# Autodesk Inventor assembly: PowerTransmission
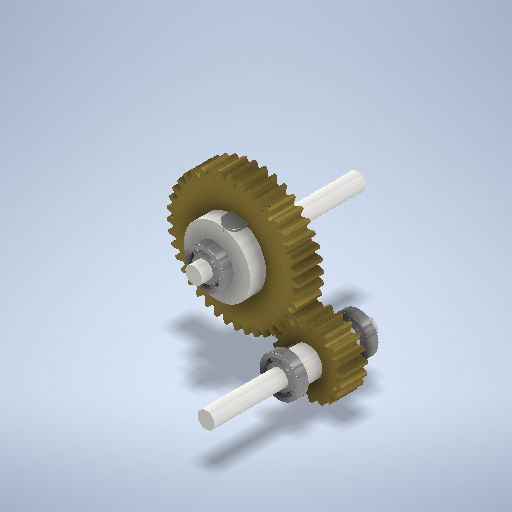
[picture p0: Inventor's stored thumbnail of the model, 512x512]
Saved by Autodesk Inventor 2025.2 (Build 292293000, 293)
## iProperties
Created: 2024-11-07
Part Number: PowerTransmission
Document SubType Name: Assembly
Designer: hongquan
Author: hongquan
## Documents named in this file (8)
- C:\Users\hongquan\Documents\GitHub\Optimal-Design-Robot\Inventor\PowerTransmission.iam
- C:\Users\hongquan\Documents\GitHub\Optimal-Design-Robot\Inventor\PowerTransmission\Design Accelerator\Spur Gears1.iam
- C:\Users\hongquan\Documents\GitHub\Optimal-Design-Robot\Inventor\PowerTransmission\Design Accelerator\Spur Gears2.iam
- C:\Users\hongquan\Documents\GitHub\Optimal-Design-Robot\Inventor\Shaft1.ipt
- C:\Users\hongquan\Documents\GitHub\Optimal-Design-Robot\Inventor\Shaft2.ipt
- C:\Users\hongquan\Documents\GitHub\Optimal-Design-Robot\Inventor\PowerTransmission\Design Accelerator\Key Connection1.iam
- C:\Users\hongquan\Documents\GitHub\Optimal-Design-Robot\Inventor\PowerTransmission\Design Accelerator\Key Connection3.iam
- C:\Users\hongquan\Documents\GitHub\Optimal-Design-Robot\Inventor\PowerTransmission\Design Accelerator\Bearing1.iam
## Components (10 placed, 4 different names)
1. Spur Gears:1 [sub-assembly]
2. Spur Gears:2 [sub-assembly] — Mate:1, Flush:1, Mate:4, Angle:2, Angle:4
3. Shaft:2 — Mate:2, Flush:1, Flush:2, Flush:3, Angle:1, Mate:5, Angle:2, Mate:11, Mate:12, Mate:13, Mate:14
4. Shaft:1 — Mate:4, Flush:2, Flush:4, Angle:3, Mate:6, Angle:4, Mate:7, Mate:8, Mate:9, Mate:10
5. Key Connection:1 [sub-assembly] — Flush:3, Angle:1, Mate:5
6. Key Connection:2 [sub-assembly] — Flush:4, Angle:3, Mate:6
7. Bearing:1 [sub-assembly] — Mate:7, Mate:8
8. Bearing:2 [sub-assembly] — Mate:11, Mate:12
9. Bearing:3 [sub-assembly] — Mate:13, Mate:14
10. Bearing:4 [sub-assembly] — Mate:9, Mate:10
## Relationships (21: Mate 13, Flush 4, Angle 4)
- Mate:1: Spur Gears:2
- Mate:2: Shaft:2
- Flush:1 (30 mm): Spur Gears:2 ↔ Shaft:2
- Mate:4: Spur Gears:2 ↔ Shaft:1
- Flush:2: Shaft:2 ↔ Shaft:1
- Flush:3: Shaft:2 ↔ Key Connection:1
- Angle:1 (355 deg): Shaft:2 ↔ Key Connection:1
- Mate:5: Shaft:2 ↔ Key Connection:1
- Angle:2 (124.6435 deg): Spur Gears:2 ↔ Shaft:2
- Flush:4 (10.1713 mm): Shaft:1 ↔ Key Connection:2
- Angle:3 (0 deg): Shaft:1 ↔ Key Connection:2
- Mate:6: Shaft:1 ↔ Key Connection:2
- Angle:4 (3.146 deg): Spur Gears:2 ↔ Shaft:1
- Mate:7: Shaft:1 ↔ Bearing:1
- Mate:8: Shaft:1 ↔ Bearing:1
- Mate:9: Shaft:1 ↔ Bearing:4
- Mate:10: Shaft:1 ↔ Bearing:4
- Mate:11: Shaft:2 ↔ Bearing:2
- Mate:12: Shaft:2 ↔ Bearing:2
- Mate:13: Shaft:2 ↔ Bearing:3
- Mate:14: Shaft:2 ↔ Bearing:3
